# Autodesk Inventor assembly: xyArmature
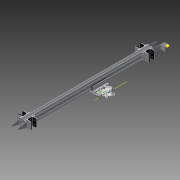
[picture p0: Inventor's stored thumbnail of the model, 180x180]
Saved by Autodesk Inventor 2013 (Build 170138000, 138)
## iProperties
Created: 2013-09-17
Part Number: xyArmature
Document SubType Name: Assembly
Designer: Ian
Mass: 4612.21 g
Surface Area: 12236.5 cm^2
Volume: 2864.57 cm^3
Density: 1.61009 g/cm^3
Author: Ian
## Documents named in this file (8)
- C:\Users\Ian\Documents\Inventor\xyPartStorage\loader\xyArmature.iam
- C:\Users\Ian\Documents\Inventor\xyPartStorage\80-20 models\high-cycle-bearing\6835.iam
- C:\Users\Ian\Documents\Inventor\xyPartStorage\80-20 models\T-slot\1530-50_5.ipt
- C:\Users\Ian\Documents\Inventor\xyPartStorage\loader\loader.iam
- C:\Users\Ian\Documents\Inventor\xyPartStorage\loader\pully mount.ipt
- C:\Users\Ian\Documents\Inventor\xyPartStorage\loader\x_motor_mount.ipt
- C:\Users\Ian\Documents\Inventor\xyPartStorage\stepper\NEMA_17.ipt
- C:\Users\Ian\Documents\Inventor\xyPartStorage\loader\x_axis_shaft_support.ipt
## Components (13 placed, 7 different names)
1. 6835:1 [sub-assembly]
2. 6835:2 [sub-assembly]
3. 1530-50_5:1
4. 6835:3 [sub-assembly]
5. 6835:4 [sub-assembly]
6. 6835:5 [sub-assembly]
7. 6835:6 [sub-assembly]
8. loader:1 [sub-assembly]
9. pully mount:1
10. pully mount:2
11. x_motor_mount:1
12. NEMA_17:1
13. x_axis_shaft_support:1
## Relationships (32: Mate 22, Flush 10)
- [Flush]: 6835:1 ↔ 6835:2
- [Flush] (-2.286 mm): 6835:1 ↔ 1530-50_5:1
- [Flush]: 6835:1 ↔ 1530-50_5:1
- [Mate]: 6835:1 ↔ 1530-50_5:1
- [Mate]: 1530-50_5:1 ↔ 6835:3
- [Mate]: 1530-50_5:1 ↔ 6835:3
- [Mate]: 6835:3 ↔ 6835:4
- [Flush]: 6835:3 ↔ 6835:4
- [Flush]: 6835:3 ↔ 6835:4
- [Mate]: 1530-50_5:1 ↔ 6835:5
- [Flush]: 1530-50_5:1 ↔ 6835:5
- [Flush]: 6835:2 ↔ 6835:5
- [Flush]: 6835:1 ↔ 6835:6
- [Mate]: 1530-50_5:1 ↔ 6835:6
- [Flush]: 1530-50_5:1 ↔ 6835:6
- [Mate]: 6835:2 ↔ 1530-50_5:1
- [Mate]: 6835:4 ↔ loader:1
- [Mate]: 6835:3 ↔ loader:1
- [Mate]: 6835:4 ↔ loader:1
- [Mate]: 6835:6 ↔ pully mount:2
- [Mate]: 6835:6 ↔ pully mount:2
- [Mate]: 6835:6 ↔ pully mount:2
- [Mate]: 6835:1 ↔ pully mount:1
- [Mate]: 6835:1 ↔ pully mount:1
- [Mate]: 6835:1 ↔ pully mount:1
- [Mate]: 6835:2 ↔ x_motor_mount:1
- [Mate]: 6835:2 ↔ x_motor_mount:1
- [Mate]: x_motor_mount:1 ↔ NEMA_17:1
- [Flush]: x_motor_mount:1 ↔ NEMA_17:1
- [Mate]: x_motor_mount:1 ↔ NEMA_17:1
- [Mate]: 6835:5 ↔ x_axis_shaft_support:1
- [Mate]: 6835:5 ↔ x_axis_shaft_support:1
